# Autodesk Inventor assembly: custodiafinal
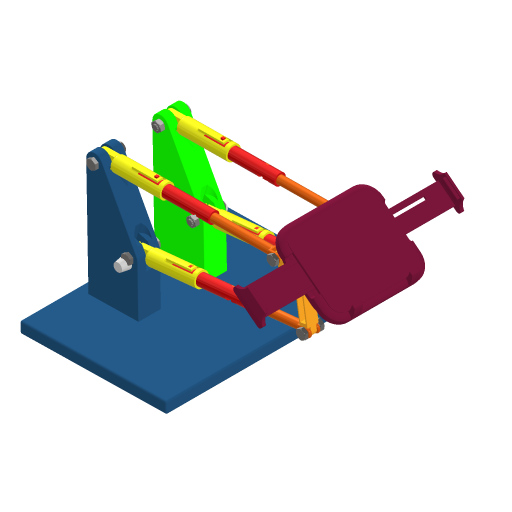
[picture p0: Inventor's stored thumbnail of the model, 512x512]
Saved by Autodesk Inventor 2024 (Build 280153000, 153)
## iProperties
Created: 2024-04-16
Part Number: custodiafinal
Document SubType Name: Assembly
Designer: alexz
Author: alexz
## Documents named in this file (21)
- C:\Users\alexz\Documents\Inventor\Esercizi\Progetto\custodiafinale.iam
- C:\Users\alexz\Documents\Inventor\Esercizi\Progetto\alettadx.ipt
- C:\Users\alexz\Documents\Inventor\Esercizi\Progetto\alettasx.ipt
- C:\Users\alexz\Documents\Inventor\Esercizi\Progetto\dietrotablet.ipt
- C:\Users\alexz\Documents\Inventor\Esercizi\Progetto\Portatablet.ipt
- C:\Users\alexz\Documents\Inventor\Esercizi\Progetto\biellaa.ipt
- C:\Users\alexz\Documents\Inventor\Esercizi\Progetto\torree.ipt
- C:\Users\alexz\Documents\Inventor\Esercizi\Progetto\base2.ipt
- C:\Users\alexz\Documents\Inventor\Esercizi\Progetto\ipad.ipt
- C:\Users\alexz\Documents\Inventor\Content Center Files\R2024\en-US\BS EN ISO 7045 H\EN ISO 7045 - M3 x 10 - 4.8 - H(1).ipt
- C:\Users\alexz\Documents\Inventor\Esercizi\Progetto\astaoscilla2_306.ipt
- C:\Users\alexz\Documents\Inventor\Esercizi\Progetto\astaoscilla3_(306).ipt
- C:\Users\alexz\Documents\Inventor\Esercizi\Progetto\asteoscila1_(306).ipt
- C:\Users\alexz\Documents\Inventor\Esercizi\Progetto\astaoscilla2_(310).ipt
- C:\Users\alexz\Documents\Inventor\Esercizi\Progetto\astaoscilla3_(301).ipt
- C:\Users\alexz\Documents\Inventor\Esercizi\Progetto\asteoscila1_(301).ipt
- C:\Users\alexz\Documents\Inventor\Esercizi\Progetto\bottone3.ipt
- C:\Users\alexz\Documents\Inventor\Esercizi\Progetto\torree3.ipt
- C:\Users\alexz\Documents\Inventor\Esercizi\Progetto\vite_magggica.ipt
- C:\Users\alexz\Documents\Inventor\Content Center Files\R2024\en-US\ISO 4032(2)\ISO 4032 - M10 - ISO.ipt
- C:\Users\alexz\Documents\Inventor\Esercizi\Progetto\vite_magggica50.ipt
## Components (44 placed, 19 different names)
1. alettadx:1 — Slider:2
2. alettasx:1 — Slider:3
3. Portatablet:1 — Rigid:1
4. biellaa:1 — Rotational:12, Rotational:14, Rigid:19
5. biellaa:2 — Rotational:15, Rotational:17, Rigid:18
6. torree:1 — Rigid:9, Rotational:13, Rotational:19, Rigid:11, Insert:15, Insert:17, Insert:19, Insert:20
7. dietrotablet:1 — Slider:2, Slider:3, Rigid:1, Cylindrical:5, Cylindrical:6, Cylindrical:7, Cylindrical:8, Rigid:18, Rigid:19
8. base2:1 — Rigid:9, Rigid:16
9. ipad:1
10. BS EN ISO 7045 H - Metric M3 x 10 - 4.8 - H:1 — Cylindrical:6
11. BS EN ISO 7045 H - Metric M3 x 10 - 4.8 - H:2 — Cylindrical:7
12. BS EN ISO 7045 H - Metric M3 x 10 - 4.8 - H:3 — Cylindrical:8
13. BS EN ISO 7045 H - Metric M3 x 10 - 4.8 - H:4 — Cylindrical:5
14. astaoscilla2_306:1 — Rigid:15, Cylindrical:4
15. astaoscilla3_(306):1 — Rotational:15, Cylindrical:4, Insert:9, Insert:13
16. asteoscila1_(306):1 — Rigid:15, Rotational:20
17. astaoscilla2_306:2 — Rigid:14, Cylindrical:3
18. astaoscilla3_(306):2 — Rotational:12, Cylindrical:3, Insert:10, Insert:14
19. asteoscila1_(306):2 — Rotational:19, Rigid:14
20. astaoscilla2_(310):1 — Rigid:13, Cylindrical:1
21. astaoscilla3_(301):1 — Rotational:14, Cylindrical:1, Insert:7, Insert:11
22. asteoscila1_(301):1 — Rotational:13, Rigid:13
23. astaoscilla2_(310):2 — Rigid:12, Cylindrical:2
24. astaoscilla3_(301):2 — Rotational:17, Cylindrical:2, Insert:8, Insert:12
25. asteoscila1_(301):2 — Rigid:12, Rotational:21
26. bottone3:1 — Rigid:11
27. torree3:1 — Rigid:16, Rotational:20, Rotational:21, Rigid:17, Insert:16, Mate:1, Insert:18, Insert:21
28. bottone3:2 — Rigid:17
29. ISO 4014 M10 x 45:1 — Insert:7
30. ISO 4014 M10 x 45:3 — Insert:9
31. ISO 4014 M10 x 45:4 — Insert:10
32. ISO 4014 M10 x 45:5 — Insert:8
33. ISO 4032 M10:1 — Insert:11
34. ISO 4032 M10:2 — Insert:12
35. ISO 4032 M10:3 — Insert:13
36. ISO 4032 M10:4 — Insert:14
37. ISO 4014 M10 x 45:6 — Insert:16
38. ISO 4014 M10 x 45:7 — Insert:15
39. ISO 4032 M10:5 — Insert:17
40. ISO 4032 M10:6 — Mate:1
41. ISO 4032 M10:7 — Insert:21
42. ISO 4032 M10:8 — Insert:20
43. ISO 4014 M10 x 45:8 — Insert:18
44. ISO 4014 M10 x 45:9 — Insert:19
## Relationships (45: Insert 15, WeldJoint 11, RevoluteJoint 8, CylindricalJoint 8, TranslationJoint 2, Mate 1)
- Slider:2 [TranslationJoint]: alettadx:1 ↔ dietrotablet:1
- Slider:3 [TranslationJoint]: alettasx:1 ↔ dietrotablet:1
- Rigid:1 [WeldJoint]: Portatablet:1 ↔ dietrotablet:1
- Rigid:9 [WeldJoint]: torree:1 ↔ base2:1
- Rotational:12 [RevoluteJoint]: biellaa:1 ↔ astaoscilla3_(306):2
- Rotational:13 [RevoluteJoint]: torree:1 ↔ asteoscila1_(301):1
- Rotational:14 [RevoluteJoint]: biellaa:1 ↔ astaoscilla3_(301):1
- Rotational:15 [RevoluteJoint]: biellaa:2 ↔ astaoscilla3_(306):1
- Rotational:17 [RevoluteJoint]: biellaa:2 ↔ astaoscilla3_(301):2
- Rotational:19 [RevoluteJoint]: torree:1 ↔ asteoscila1_(306):2
- Rigid:11 [WeldJoint]: torree:1 ↔ bottone3:1
- Rigid:12 [WeldJoint] (45.298 mm): astaoscilla2_(310):2 ↔ asteoscila1_(301):2
- Rigid:13 [WeldJoint] (45.298 mm): astaoscilla2_(310):1 ↔ asteoscila1_(301):1
- Rigid:14 [WeldJoint] (45.284 mm): astaoscilla2_306:2 ↔ asteoscila1_(306):2
- Rigid:15 [WeldJoint] (45.284 mm): astaoscilla2_306:1 ↔ asteoscila1_(306):1
- Cylindrical:1: astaoscilla2_(310):1 ↔ astaoscilla3_(301):1
- Cylindrical:2: astaoscilla2_(310):2 ↔ astaoscilla3_(301):2
- Cylindrical:3: astaoscilla2_306:2 ↔ astaoscilla3_(306):2
- Cylindrical:4: astaoscilla2_306:1 ↔ astaoscilla3_(306):1
- Rigid:16 [WeldJoint]: base2:1 ↔ torree3:1
- Rotational:20 [RevoluteJoint]: asteoscila1_(306):1 ↔ torree3:1
- Rotational:21 [RevoluteJoint]: asteoscila1_(301):2 ↔ torree3:1
- Rigid:17 [WeldJoint]: torree3:1 ↔ bottone3:2
- Cylindrical:5: dietrotablet:1 ↔ BS EN ISO 7045 H - Metric M3 x 10 - 4.8 - H:4
- Cylindrical:6: dietrotablet:1 ↔ BS EN ISO 7045 H - Metric M3 x 10 - 4.8 - H:1
- Cylindrical:7: dietrotablet:1 ↔ BS EN ISO 7045 H - Metric M3 x 10 - 4.8 - H:2
- Cylindrical:8: dietrotablet:1 ↔ BS EN ISO 7045 H - Metric M3 x 10 - 4.8 - H:3
- Rigid:18 [WeldJoint]: biellaa:2 ↔ dietrotablet:1
- Rigid:19 [WeldJoint]: biellaa:1 ↔ dietrotablet:1
- Insert:7: astaoscilla3_(301):1 ↔ ISO 4014 M10 x 45:1
- Insert:8: astaoscilla3_(301):2 ↔ ISO 4014 M10 x 45:5
- Insert:9: astaoscilla3_(306):1 ↔ ISO 4014 M10 x 45:3
- Insert:10: astaoscilla3_(306):2 ↔ ISO 4014 M10 x 45:4
- Insert:11: astaoscilla3_(301):1 ↔ ISO 4032 M10:1
- Insert:12: astaoscilla3_(301):2 ↔ ISO 4032 M10:2
- Insert:13: astaoscilla3_(306):1 ↔ ISO 4032 M10:3
- Insert:14: astaoscilla3_(306):2 ↔ ISO 4032 M10:4
- Insert:15: torree:1 ↔ ISO 4014 M10 x 45:7
- Insert:16: torree3:1 ↔ ISO 4014 M10 x 45:6
- Insert:17: torree:1 ↔ ISO 4032 M10:5
- Mate:1: torree3:1 ↔ ISO 4032 M10:6
- Insert:18: torree3:1 ↔ ISO 4014 M10 x 45:8
- Insert:19: torree:1 ↔ ISO 4014 M10 x 45:9
- Insert:20: torree:1 ↔ ISO 4032 M10:8
- Insert:21: torree3:1 ↔ ISO 4032 M10:7
